# Autodesk Inventor assembly: MUXAssembly1
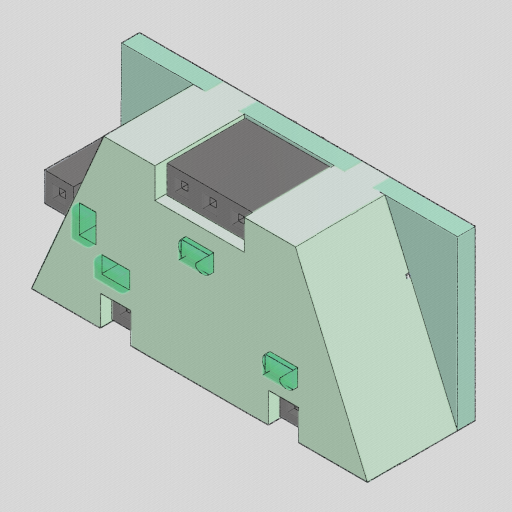
[picture p0: Inventor's stored thumbnail of the model, 512x512]
Saved by Autodesk Inventor 2024.3 (Build 283343000, 343)
## iProperties
Created: 2024-03-15
Part Number: MUXAssembly1
Document SubType Name: Assembly
Designer: Jonat
Author: Jonat
## Documents named in this file (5)
- C:\Git\DigitalLogicProject\Models\MUX\MUXAssembly1.iam
- C:\Git\DigitalLogicProject\Models\LIGHTPIPING\LightPipe.ipt
- C:\Git\DigitalLogicProject\Models\MUX\MUX.ipt
- C:\Git\DigitalLogicProject\Models\MUX\MUXPCB.ipt
- C:\Git\DigitalLogicProject\Models\LIGHTPIPING\LightPipeThin.ipt
## Components (6 placed, 4 different names)
1. LightPipe:1 — Mate:8, Mate:9, Mate:10
2. LightPipeThin:1 — Mate:14
3. LightPipeThin:2
4. LightPipe:4 — Mate:11, Mate:12, Mate:13
5. MUX:1 — Flush:1, Mate:8, Mate:9, Mate:11, Mate:12, Mate:14, Flush:2, Mate:15, Mate:16, Mate:17
6. MUXPCB:1 — Flush:1, Mate:10, Mate:13, Flush:2, Mate:15, Mate:16, Mate:17
## Relationships (16: Mate 14, Flush 2)
- [Mate]: LightPipeThin:1 ↔ MUX:1
- [Mate]: LightPipeThin:1 ↔ MUX:1
- [Mate]: LightPipeThin:2 ↔ MUX:1
- [Mate]: LightPipeThin:2 ↔ MUX:1
- Flush:1: MUX:1 ↔ MUXPCB:1
- Mate:8: LightPipe:1 ↔ MUX:1
- Mate:9: LightPipe:1 ↔ MUX:1
- Mate:10: LightPipe:1 ↔ MUXPCB:1
- Mate:11: LightPipe:4 ↔ MUX:1
- Mate:12: LightPipe:4 ↔ MUX:1
- Mate:13: LightPipe:4 ↔ MUXPCB:1
- Mate:14: LightPipeThin:1 ↔ MUX:1
- Flush:2: MUX:1 ↔ MUXPCB:1
- Mate:15: MUX:1 ↔ MUXPCB:1
- Mate:16: MUX:1 ↔ MUXPCB:1
- Mate:17: MUX:1 ↔ MUXPCB:1
